# Autodesk Inventor assembly: 新型３クランクアセンブリ
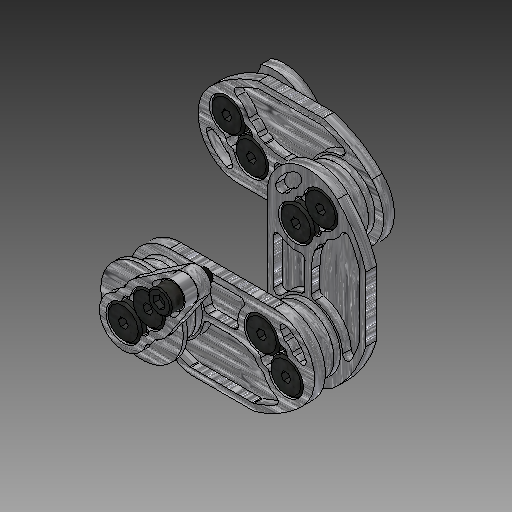
[picture p0: Inventor's stored thumbnail of the model, 512x512]
Saved by Autodesk Inventor 2019 (Build 230136000, 136)
## iProperties
Created: 2019-04-15
Part Number: 新型３クランクアセンブリ
Material: 一般
Document SubType Name: Assembly
Designer: tanjihayato
Mass: 33.8009 g
Surface Area: 150.388 cm^2
Volume: 9.40711 cm^3
Density: 3.59312 g/cm^3
Author: tanjihayato
## Documents named in this file (8)
- \\Mac\Home\Documents\Inventor\2019お遊び機体\新型３クランクアセンブリ.iam
- \\Mac\Home\Documents\Inventor\2019お遊び機体\新型３クランク.ipt
- \\Mac\Home\Documents\Inventor\2019お遊び機体\新型３脚カム.ipt
- \\Mac\Home\Documents\Inventor\2019お遊び機体\新型３クランク根本.ipt
- \\Mac\Home\Documents\Inventor\2019お遊び機体\新型３涙.ipt
- \\Mac\Home\Documents\Inventor\2019お遊び機体\低頭ねじM4×8.ipt
- \\Mac\Home\Documents\Inventor\2019お遊び機体\スペーサ　m3-l3.ipt
- \\Mac\Home\Documents\Inventor\2019お遊び機体\キャップボルトM3×8.ipt
## Components (19 placed, 7 different names)
1. 新型３クランク:1 — 挿入:1, メイト:1, 挿入:7, メイト:7, 挿入:9, 挿入:10
2. 新型３クランク:2 — 挿入:2, メイト:2, 挿入:6, メイト:6, 挿入:13, 挿入:14
3. 新型３クランク:3 — 挿入:3, メイト:3, 挿入:5, メイト:5, 挿入:15, 挿入:16
4. 新型３脚カム:1 — 挿入:1, メイト:1, 挿入:8, メイト:8
5. 新型３脚カム:2 — 挿入:2, メイト:2, 挿入:7, メイト:7
6. 新型３脚カム:3 — 挿入:3, メイト:3, 挿入:6, メイト:6
7. 新型３脚カム:4 — 挿入:4, メイト:4, 挿入:5, メイト:5
8. 新型３クランク根本:1 — 挿入:4, メイト:4
9. 新型３涙:1 — 挿入:8, メイト:8, 挿入:11, 挿入:12, 挿入:17
10. 低頭ねじM4×8:1 — 挿入:9
11. 低頭ねじM4×8:2 — 挿入:10
12. 低頭ねじM4×8:3 — 挿入:11
13. 低頭ねじM4×8:4 — 挿入:12
14. 低頭ねじM4×8:5 — 挿入:14
15. 低頭ねじM4×8:6 — 挿入:13
16. 低頭ねじM4×8:7 — 挿入:15
17. 低頭ねじM4×8:8 — 挿入:16
18. スペーサ　m3-l3:1 — 挿入:17, 挿入:18
19. キャップボルトM3×8:1 — 挿入:18
## Relationships (26: Insert 18, Mate 8)
- 挿入:1 [Insert]: 新型３クランク:1 ↔ 新型３脚カム:1
- メイト:1 [Mate]: 新型３クランク:1 ↔ 新型３脚カム:1
- 挿入:2 [Insert]: 新型３クランク:2 ↔ 新型３脚カム:2
- メイト:2 [Mate]: 新型３クランク:2 ↔ 新型３脚カム:2
- 挿入:3 [Insert]: 新型３クランク:3 ↔ 新型３脚カム:3
- メイト:3 [Mate]: 新型３クランク:3 ↔ 新型３脚カム:3
- 挿入:4 [Insert]: 新型３脚カム:4 ↔ 新型３クランク根本:1
- メイト:4 [Mate]: 新型３脚カム:4 ↔ 新型３クランク根本:1
- 挿入:5 [Insert]: 新型３クランク:3 ↔ 新型３脚カム:4
- メイト:5 [Mate]: 新型３クランク:3 ↔ 新型３脚カム:4
- 挿入:6 [Insert]: 新型３クランク:2 ↔ 新型３脚カム:3
- メイト:6 [Mate]: 新型３クランク:2 ↔ 新型３脚カム:3
- 挿入:7 [Insert]: 新型３クランク:1 ↔ 新型３脚カム:2
- メイト:7 [Mate]: 新型３クランク:1 ↔ 新型３脚カム:2
- 挿入:8 [Insert]: 新型３脚カム:1 ↔ 新型３涙:1
- メイト:8 [Mate]: 新型３脚カム:1 ↔ 新型３涙:1
- 挿入:9 [Insert]: 新型３クランク:1 ↔ 低頭ねじM4×8:1
- 挿入:10 [Insert]: 新型３クランク:1 ↔ 低頭ねじM4×8:2
- 挿入:11 [Insert]: 新型３涙:1 ↔ 低頭ねじM4×8:3
- 挿入:12 [Insert]: 新型３涙:1 ↔ 低頭ねじM4×8:4
- 挿入:13 [Insert]: 新型３クランク:2 ↔ 低頭ねじM4×8:6
- 挿入:14 [Insert]: 新型３クランク:2 ↔ 低頭ねじM4×8:5
- 挿入:15 [Insert]: 新型３クランク:3 ↔ 低頭ねじM4×8:7
- 挿入:16 [Insert]: 新型３クランク:3 ↔ 低頭ねじM4×8:8
- 挿入:17 [Insert]: 新型３涙:1 ↔ スペーサ　m3-l3:1
- 挿入:18 [Insert]: スペーサ　m3-l3:1 ↔ キャップボルトM3×8:1
